# Autodesk Inventor assembly: Assembly1
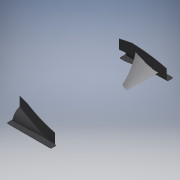
[picture p0: Inventor's stored thumbnail of the model, 180x180]
Saved by Autodesk Inventor 2018.1 (Build 221171000, 171)
## iProperties
Created: 2017-10-30
Part Number: Assembly1
Material: 一般
Document SubType Name: Assembly
Designer: ku_sk
Author: ku_sk
## Documents named in this file (6)
- D:\kuwano\Documents\Inventor\KITformula\KS-15_Aero_CAD\test\Assembly1.iam
- D:\kuwano\Documents\Inventor\KITformula\KS-15_Aero_CAD\test\test_front_end_plate.ipt
- D:\kuwano\Documents\Inventor\KITformula\KS-15_Aero_CAD\test\test_front_element_1.ipt
- D:\kuwano\Documents\Inventor\KITformula\KS-15_Aero_CAD\test\test_front_element_2.ipt
- D:\kuwano\Documents\Inventor\KITformula\KS-15_Aero_CAD\test\test_front_element_3.ipt
- D:\kuwano\Documents\Inventor\KITformula\KS-15_Aero_CAD\test\test_front_end_plate_MIR.ipt
## Components (5 placed, 5 different names)
1. test_front_end_plate:1 — フラッシュ:1, フラッシュ:2, メイト:1
2. test_front_element_1:1
3. test_front_element_2:1
4. test_front_element_3:1
5. test_front_end_plate_MIR:1 — フラッシュ:1, フラッシュ:2, メイト:1
## Relationships (3: Flush 2, Mate 1)
- フラッシュ:1 [Flush]: test_front_end_plate:1 ↔ test_front_end_plate_MIR:1
- フラッシュ:2 [Flush]: test_front_end_plate:1 ↔ test_front_end_plate_MIR:1
- メイト:1 [Mate] (1000 mm): test_front_end_plate:1 ↔ test_front_end_plate_MIR:1
